# Autodesk Inventor assembly: Assembly_Cube_Lens_holder_v3
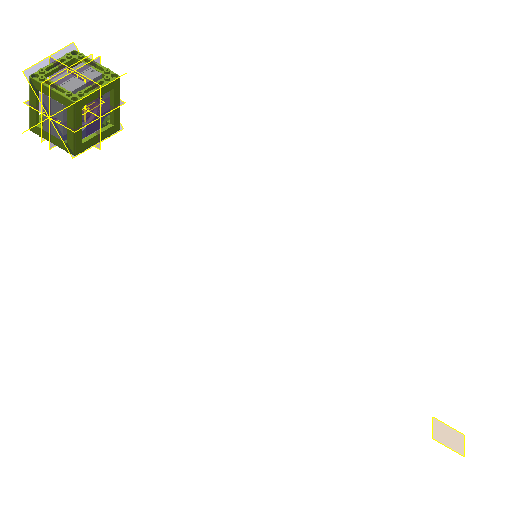
[picture p0: Inventor's stored thumbnail of the model, 512x512]
Saved by Autodesk Inventor 2023 (Build 270158000, 158)
## iProperties
Created: 2020-11-11
Part Number: Assembly_Cube_Lens_holder_v3
Document SubType Name: Assembly
Designer: marsikovabarbora
Author: marsikovabarbora
## Documents named in this file (6)
- C:\Users\diederichbenedict\Downloads\UC2 setup design\UC2 setup design\Assembly_Cube_Thorlabs_Cage_v3.iam
- C:\Users\diederichbenedict\Downloads\UC2 setup design\UC2 setup design\Assembly_Cube_empty_IM_v3.iam
- C:\Users\diederichbenedict\Downloads\UC2 setup design\UC2 setup design\00_Thorlabs_Cage_CP33_M.ipt
- C:\Users\diederichbenedict\Downloads\UC2 setup design\UC2 setup design\20_Cube_Insert_Thorlabs_Pins.ipt
- C:\Users\diederichbenedict\Downloads\UC2 setup design\UC2 setup design\00_THORLABS_AC254-050-A-ML-Step.ipt
- C:\Users\diederichbenedict\Downloads\UC2 setup design\UC2 setup design\20_Cube_Insert_Thorlabs_SM1Tube.ipt
## Components (5 placed, 5 different names)
1. Assembly_Cube_empty_IM_v3:1 [sub-assembly] — Mate:1, Mate:2, Mate:3, Passend:4, Passend:5, Passend:13, Winkel:1
2. 00_Thorlabs_Cage_CP33_M:1
3. 20_Cube_Insert_Thorlabs_Pins:1 — Passend:4, Passend:5
4. 20_Cube_Insert_Thorlabs_SM1Tube:1 — Mate:10, Mate:11, Mate:12, Passend:13, Winkel:1
5. 00_THORLABS_AC254-050-A-ML-Step:1 — Mate:11, Mate:12
## Relationships (10: Mate 9, Angle 1)
- Mate:1: Assembly_Cube_empty_IM_v3:1
- Mate:2: Assembly_Cube_empty_IM_v3:1
- Mate:3: Assembly_Cube_empty_IM_v3:1
- Passend:4 [Mate]: Assembly_Cube_empty_IM_v3:1 ↔ 20_Cube_Insert_Thorlabs_Pins:1
- Passend:5 [Mate]: Assembly_Cube_empty_IM_v3:1 ↔ 20_Cube_Insert_Thorlabs_Pins:1
- Mate:10: 20_Cube_Insert_Thorlabs_SM1Tube:1
- Mate:11: 20_Cube_Insert_Thorlabs_SM1Tube:1 ↔ 00_THORLABS_AC254-050-A-ML-Step:1
- Mate:12: 20_Cube_Insert_Thorlabs_SM1Tube:1 ↔ 00_THORLABS_AC254-050-A-ML-Step:1
- Passend:13 [Mate]: Assembly_Cube_empty_IM_v3:1 ↔ 20_Cube_Insert_Thorlabs_SM1Tube:1
- Winkel:1 [Angle] (180 deg): Assembly_Cube_empty_IM_v3:1 ↔ 20_Cube_Insert_Thorlabs_SM1Tube:1
